# Autodesk Inventor assembly: Assembly2
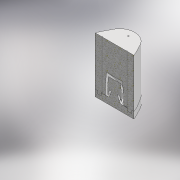
[picture p0: Inventor's stored thumbnail of the model, 180x180]
Saved by Autodesk Inventor 2021 (Build 250183000, 183)
## iProperties
Created: 2020-06-24
Part Number: Assembly2
Document SubType Name: Assembly
Designer: Derm
Author: Derm
## Documents named in this file (3)
- C:\Users\Derm\n95\v7\maskBodyV4Molds\Assembly2.iam
- C:\Users\Derm\n95\v7\maskBodyV4Molds\mainLower.ipt
- C:\Users\Derm\n95\v7\maskBodyV4Molds\upper.ipt
## Components (2 placed, 2 different names)
1. mainLower:1 — Flush:1, Flush:2, Flush:3
2. upper:1 — Flush:1, Flush:2, Flush:3
## Relationships (3: Flush 3)
- Flush:1: mainLower:1 ↔ upper:1
- Flush:2: mainLower:1 ↔ upper:1
- Flush:3: mainLower:1 ↔ upper:1
